# Autodesk Inventor assembly: Chassis_Wheel_AndyMark_am-0420
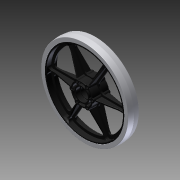
[picture p0: Inventor's stored thumbnail of the model, 180x180]
Saved by Autodesk Inventor 2011 (Build 150239000, 239)
## iProperties
Category: Drive Train
Company: Autodesk Inc.
Created: 2009-12-04
Part Number: Chassis_Wheel_AndyMark_am-0420
Document SubType Name: Assembly
Designer: Autodesk Inc.
Catalog Web Link: http://andymark.biz
Description: 2010 FIRST wheel, plastic tread
Vendor: AndyMark
Author: Autodesk Inc.
## Documents named in this file (3)
- C:\Data Folder\FIRST KOP 2011\All Parts\Chassis\Chassis_Wheel_AndyMark_am-0420.iam
- C:\Data Folder\FIRST KOP 2011\All Parts\Drive Train\DriveTrain_WheelRim_AndyMark_am-0284.ipt
- C:\Data Folder\FIRST KOP 2011\All Parts\Drive Train\DriveTrain_WheelTread_AndyMark_am-0284.ipt
## Components (2 placed, 2 different names)
1. DriveTrain_WheelRim_AndyMark_am-0420:1 — Mate:1, Flush:1
2. DriveTrain_WheelTread_AndyMark_am-0420:1 — Mate:1, Flush:1
## Relationships (2: Mate 1, Flush 1)
- Mate:1: DriveTrain_WheelRim_AndyMark_am-0420:1 ↔ DriveTrain_WheelTread_AndyMark_am-0420:1
- Flush:1: DriveTrain_WheelRim_AndyMark_am-0420:1 ↔ DriveTrain_WheelTread_AndyMark_am-0420:1
